# Autodesk Inventor assembly: Pneumatic piston
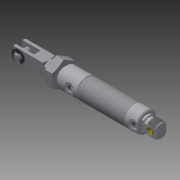
[picture p0: Inventor's stored thumbnail of the model, 180x180]
Saved by Autodesk Inventor 2015 (Build 190159000, 159)
## iProperties
Category: PARTsolutions
Company: BIMBA
Created: 2015-01-25
Part Number: Pneumatic piston
Catalog Web Link: www.cadenas.de
Description: Original Line Standard Air Cylinders-
Vendor: BIMBA
Document SubType Name: Assembly
Designer: chapale16
Manufacturer: BIMBA
PSOL_IDENT_0: {$CADENAS_DATA\23d-libs\bimba\bimba\bimba_imperial\bimba_full_line\original_line_cylinders\standard_
PSOL_IDENT_1: air_cylinders\standard_air_cylinder_asmtab.prj},327 {VTYP=3D},{STYP=ASSTAB},{NB=020.5-DXP(F,D-850)},
PSOL_IDENT_2: {LINA=020.5-DXP},{NN=Original Line Standard Air Cylinders},{DATE=08.09.2014 04:47:41},{GEOMDATE=08.0
PSOL_IDENT_3: 9.2014 04:47:39},{VERSION=},{LINEID=40},{LINESUBID=-1},{WBVAR=STROKE,ACTING,MNT,DER,NR,BM,CO,OO,VO,M
PSOL_IDENT_4: ,EE,EEL,K,Q,Y,G,T,B,H,SER,SR,NT,W,HL,STPT1,STPT2,STPT3,STPT4,MB,PB,PRC,TB,MN}  {NB=020.5-DXP(F,D-850
PSOL_IDENT_5: )},{LINA=020.5-DXP},{KT=DUMMY},{PN=020.5-DXP},{PNC=020.5-DXP(F,D-850)},{PNA=(D-850)},{DASH=-},{BORE1=
PSOL_IDENT_6: 0.56250000},{BORE=9/16\" (02)},{BOREPN=02},{STROKE=0.500},{STROKEALG=[0.011:50/0.001]},{STROKE1=0.50
PSOL_IDENT_7: 0},{ACTING=D},{ACTINGALG= '' , 'Single Acting (SA)' , 'R' , 'Reverse Single Acting (SA)' , 'D' , 'Do
PSOL_IDENT_8: uble Acting (SA)' },{ACTINGPN=D},{MNT=XP},{MNTALG= '' , 'Front Nose Mounting (SA)' , 'XP' , 'Double
PSOL_IDENT_9: End or Rear Pivot Mounting (SA)' , 'X' , 'Double End Mounting (SA)' },{TYPE=},{MNTPN=XP},{DER=},{DER
PSOL_IDENT_10: ALG= '' , 'N/A' },{NR=},{NRALG= '' , 'N/A' },{NRPN=},{BM=},{BMALG= '' , 'N/A' },{BMPN=},{CO=},{COALG=
PSOL_IDENT_11: '' , 'N/A' },{OO=},{OOALG= '', 'N/A' },{OOPN=},{VO=Z},{VOALG= 'Z' , 'N/A' },{VOPN=},{OOVOPN=},{M=},
PSOL_IDENT_12: {MALG= '', 'Without Magnet', 'M', 'With Magnet' },{EE=},{EEL=0.000},{EEMAX=49.5000},{EEALG= '', 'Wit
PSOL_IDENT_13: hout Extra Extension', 'EE', 'With Extra Extension' },{EELALG=0},{EEPN=},{EEPN1=0.000},{K=},{KALG= ''
PSOL_IDENT_14: , 'Standard' , 'K' , 'Ports Rotated 90deg K' },{KPN=},{Q=},{QALG= '' , 'N/A' },{QPN=},{Y=},{YALG= ''
PSOL_IDENT_15: , 'With Pivot Bushing' },{YPN=},{YCON=Y},{F=},{FALG= '', 'Non-Coated (Standard)', 'F', 'Molycoated'
PSOL_IDENT_16: },{FPN=},{G=},{GPN=},{GPN99=},{T=},{TALG= '' , 'Standard -20° to 200°F (-29° to 95°C)' , 'N' , 'Low
PSOL_IDENT_17: Temperature' , 'V' , 'High Temperature' },{NPN=},{VPN=},{B=},{BALG= '', 'W/out Bumpers' , 'B' , 'W/
PSOL_IDENT_18: Bumpers' },{BPN=},{H=},{HALG= '', 'N/A' },{HPN=},{SER=},{SERALG= '' , 'Without Spring Extend/Return'
PSOL_IDENT_19: , 'JS' , 'With Spring Return' , 'JR' , 'With Spring Extend' },{SR=},{SRALG= '' , 'Standard Stainles
PSOL_IDENT_20: s Steel' },{SRPN=},{SRCON=0},{NT=},{NTPN=},{W=},{WALG= '' , 'Without Wiper' , 'W' , 'With Wiper' },{
PSOL_IDENT_21: WPN=},{E=},{EALG= '' , 'Standard Seals/Lube' , 'E' , 'Non-Lube Seals/Lube' },{EPN=},{HL=},{HLALG= ''
PSOL_IDENT_22: , 'Without Low Pressure Hydraulic' , 'HL' , 'With Low Pressure Hydraulic' },{ST=},{STALG= '' , 'N/A'
PSOL_IDENT_23: },{STPT1=},{STPT1ALG= '' , 'N/A' },{STPT2=},{STPT2ALG= '' , 'N/A' },{STPT3=},{STPT3ALG= '' , 'N/A'
PSOL_IDENT_24: },{STPT4=},{STPT4ALG= '' , 'N/A' },{STPN=},{MB=},{MBALG= '' , 'Without Mounting Bracket' , 'F,D-770'
PSOL_IDENT_25: , 'D-770 (front)'  , 'R,D-770' , 'D-770 (rear)' , '2x,D-770' , 'D-770 (front & rear)'},{MBPN=},{MBP
PSOL_IDENT_26: NALL=D-770},{MBPNALLREAR=D-770},{PB=},{PBALG= '' , 'Without Pivot Bracket' , 'D-12321-A' , 'D-12321-
PSOL_IDENT_27: A' },{PBPN=},{PBPNALL=D-12321-A},{PRC=F,D-850},{PRCALG= '' , 'W/out Pivot Rod Clevis' , 'F,D-850' , '
PSOL_IDENT_28: D-850 (front)' },{PRCPN=(F,D-850)},{PRCPNALL=D-850},{TB=},{TBALG= '' , 'N/A' },{TBPN=},{TBPNALL=},{M
PSOL_IDENT_29: N=},{MNALG= '' , 'N/A' },{MNPN=},{MNCONF=},{MNCONR=},{TLEN=1.3870},{FRAC=2.5600},{RGCON=},{RGDACCON=
PSOL_IDENT_30: R},{RHCON=P},{RHCON1=P},{RHCONON=1},{RHACCON=R},{FNUTCON=1},{RNUTCON=1},{FNUTPN=D-154},{RNUTPN=D-154
PSOL_IDENT_31: },{FNUTTRANS=0.0000},{RNUTTRANS=0.0000},{VHOLECON=0},{A1=1.1560},{A1N=1.0310},{A1P=1.1560},{A1B=0.00
PSOL_IDENT_32: 00},{A4=0.1570},{A4N=0.5310},{A4P=0.1570},{A5=0.0250},{A1H=0.969},{A1NH=0.5000},{A1PH=0.9690},{A1BH=
PSOL_IDENT_33: 0.0000},{A1SH=0.0000},{A2H=0.1570},{A2NH=0.1570},{LENGTH=2.5600},{LENGTH1=2.5600},{LENGTH2=2.6100},{
PSOL_IDENT_34: MUL=0.5000},{MUL11=0.5000},{MUL22=1.315},{MUL33=0.8150},{MUL2=0.5000},{MUL211=0.5000},{MUL222=2.6300
PSOL_IDENT_35: },{MUL233=1.6300},{SSS=0.5000},{RGLEN=1.0240},{RHLEN=0.6490},{SSS1=1.0000},{A13=0.7810},{DIF=0.0000}
PSOL_IDENT_36: ,{G5=0.0000},{ON=0},{SSADD=0.0000},{BADD=0.0000},{MADD=0.0000},{NVADD=0.0000},{TRACKL=1.0870},{TRACK
PSOL_IDENT_37: CON=D-74168},{TRIMCON=0},{TRIMCON1=0},{PINCON=},{FSPACE=0.4863},{SPACE=0.0362},{TEXT=0.0633},{S1=0.0
PSOL_IDENT_38: 000},{D1=0.0000},{D1N=0.6150},{D1B=0.6150},{D1P=0.0000},{FA=0.690},{RA=0.6900},{PPATH=standard_air_c
PSOL_IDENT_39: ylinder_asmtpl.prj},{MATALGHTML=<b>Standard Original Line:</b><dl><dt>Rod:</dt><dd>- Stainless Steel
PSOL_IDENT_40: </dd><dd>&nbsp;&nbsp;(5/16 9/16 Bores)</dd><dd>- High Strength Carbon Steel</dd><dd>&nbsp;&nbsp;(3/4
PSOL_IDENT_41: 3 Bore)</dd><dd>- Stainless Steel</dd><dd>&nbsp;&nbsp;(X style DXP/DX/DXDE)</dd><dt>Bearings:</dt><
PSOL_IDENT_42: dd>- Sintered Bronze</dd><dt>Body:</dt><dd>- 304 Stainless Steel</dd><dt>End Caps:</dt><dd>- Aluminu
PSOL_IDENT_43: m</dd><dt>Seals:</dt><dd>- Buna N</dd></dl>},{ASSCFGPRA=02DXP},{MBPNA=},{MNPNA=},{PRCPNA=(D-850)},{A
PSOL_IDENT_44: SSOPTACC=STPT4},{A=3.06},{HADD=0.0000},{WFL=0},{QADD=0.000},{QADD1=0.030},{TEST=0.0000},{MNTB=},{STD
PSOL_IDENT_45: NUTF=1},{STDNUTR=1}
NN: Original Line Standard Air Cylinders
NT: Standard Male Thread
NB: 020.5-DXP(F,D-850)
NBSYN: $PNC.
LINA: 020.5-DXP
PN: 020.5-DXP
PNA: (D-850)
BORE: 9/16" [02]
STROKE: 0.500
ACTING: Double [D]
MNT: Universal Double End or Rear Pivot [XP]
DER: N/A
NR: N/A
BM: N/A
CO: N/A
OO: N/A
VO: N/A
M: Without Magnet Piston
EE: Standard Rod Extension
EEL: 0.000
K: Standard
Q: N/A
Y: Pivot Bushing [Y]
G: Standard Grease Lube
T: Standard -20° to 200°F (-29° to 95°C)
B: Without Bumpers
H: N/A
SER: Without Failsafe Spring Extend/Return
SR: Standard Stainless Steel
W: Without Wiper
HL: Standard 250 PSI Air
STPT1: N/A
STPT2: N/A
STPT3: N/A
STPT4: N/A
MB: Without Mounting Bracket
PB: Without Pivot Bracket
PRC: D-850 (front)
TB: N/A
MN: N/A
A: 3.06
SUPPLIER: BIMBA
ARTICLENO: 020.5-DXP(F,D-850)
BOMINFO: 020.5-DXP
CREATOR: CADENAS GmbH
Title: 020.5-DXP
Author: Cadenas PARTsolutions
## Documents named in this file (13)
- \\lhssvr02\Homedirs\Robotics Club\CAD Model 2015\Elevator parts\Pneumatic piston.iam
- C:\Users\chapale16\Documents\020_5-DXP(F,D-850)0000_0_dummy.ipt
- C:\Users\chapale16\Documents\02R000-0_rod_guide.ipt
- C:\Users\chapale16\Documents\02R-1_3870.ipt
- C:\Users\chapale16\Documents\02P0Y000_rear_head.ipt
- C:\Users\chapale16\Documents\D-154.ipt
- C:\Users\chapale16\Documents\D-8597.ipt
- C:\Users\chapale16\Documents\020_5-DXP0_rod.ipt
- C:\Users\chapale16\Documents\D-850-dummy.ipt
- C:\Users\chapale16\Documents\D-14043.ipt
- C:\Users\chapale16\Documents\D-12304.ipt
- C:\Users\chapale16\Documents\D-5406.ipt
- C:\Users\chapale16\Documents\D-5288.ipt
## Components (13 placed, 12 different names)
1. 020_5-DXP(F,D-850)0000_0_dummy:1 — dummy_XY@1 <-> rod_guide_XY@2, dummy_Z@1 <-> rod_guide_Z@2, dummy_YZ@1 <-> rod_guide_YZ@2
2. 02R000-0_rod_guide:1 — dummy_XY@1 <-> rod_guide_XY@2, dummy_Z@1 <-> rod_guide_Z@2, dummy_YZ@1 <-> rod_guide_YZ@2, to_tube_XY@2 <-> tube_front_XY@3, to_tube_Z@2 <-> tube_front_Z@3, to_tube_YZ@2 <-> tube_front_YZ@3, to_nut_XY@2 <-> NUT_XY@7, to_nut_Z@2 <-> NUT_Z@7, to_nut_YZ@2 <-> NUT_YZ@7, to_rod_XY@2 <-> rod_cp_XY@8, to_rod_Z@2 <-> rod_cp_Z@8
3. 02R-1_3870:1 — to_tube_XY@2 <-> tube_front_XY@3, to_tube_Z@2 <-> tube_front_Z@3, to_tube_YZ@2 <-> tube_front_YZ@3, tube_rear_XY@3 <-> to_tube_XY@4, tube_rear_Z@3 <-> to_tube_Z@4, tube_rear_YZ@3 <-> to_tube_YZ@4
4. 02P0Y000_rear_head:1 — tube_rear_XY@3 <-> to_tube_XY@4, tube_rear_Z@3 <-> to_tube_Z@4, tube_rear_YZ@3 <-> to_tube_YZ@4, to_pin_XY@4 <-> bushing_XY@6, to_pin_Z@4 <-> bushing_Z@6, to_pin_YZ@4 <-> bushing_YZ@6
5. D-8597:1 — to_pin_XY@4 <-> bushing_XY@6, to_pin_Z@4 <-> bushing_Z@6, to_pin_YZ@4 <-> bushing_YZ@6
6. D-154:2 — to_nut_XY@2 <-> NUT_XY@7, to_nut_Z@2 <-> NUT_Z@7, to_nut_YZ@2 <-> NUT_YZ@7
7. 020_5-DXP0_rod:1 — to_rod_XY@2 <-> rod_cp_XY@8, to_rod_Z@2 <-> rod_cp_Z@8, to_rod_clevis_XY@8 <-> to_cyl_XY@9, to_rod_clevis_Z@8 <-> to_cyl_Z@9, to_rod_clevis_YZ@8 <-> to_cyl_YZ@9
8. D-850-dummy:1 — to_rod_clevis_XY@8 <-> to_cyl_XY@9, to_rod_clevis_Z@8 <-> to_cyl_Z@9, to_rod_clevis_YZ@8 <-> to_cyl_YZ@9, dummy_XY@9 <-> dummy_XY@10, dummy_Z@9 <-> dummy_Z@10, dummy_YZ@9 <-> dummy_YZ@10
9. D-14043:1 — dummy_XY@9 <-> dummy_XY@10, dummy_Z@9 <-> dummy_Z@10, dummy_YZ@9 <-> dummy_YZ@10, rod_clevis_body_XY@10 <-> pin_XY@11, rod_clevis_body_Z@10 <-> pin_Z@11, piston_rod_clevis_XY@10 <-> NUT_XY@14, piston_rod_clevis_Z@10 <-> NUT_Z@14
10. D-12304:1 — rod_clevis_body_XY@10 <-> pin_XY@11, rod_clevis_body_Z@10 <-> pin_Z@11, rr1_XY@11 <-> RR_XY@12, rr1_Z@11 <-> RR_Z@12, rr2_XY@11 <-> RR_XY@13, rr2_Z@11 <-> RR_Z@13
11. D-5406:1 — rr1_XY@11 <-> RR_XY@12, rr1_Z@11 <-> RR_Z@12
12. D-5406:2 — rr2_XY@11 <-> RR_XY@13, rr2_Z@11 <-> RR_Z@13
13. D-5288:1 — piston_rod_clevis_XY@10 <-> NUT_XY@14, piston_rod_clevis_Z@10 <-> NUT_Z@14
## Relationships (31: Mate 18, Angle 7, Flush 6)
- dummy_XY@1 <-> rod_guide_XY@2 [Flush]: 020_5-DXP(F,D-850)0000_0_dummy:1 ↔ 02R000-0_rod_guide:1
- dummy_Z@1 <-> rod_guide_Z@2 [Mate]: 020_5-DXP(F,D-850)0000_0_dummy:1 ↔ 02R000-0_rod_guide:1
- dummy_YZ@1 <-> rod_guide_YZ@2 [Angle] (0 deg): 020_5-DXP(F,D-850)0000_0_dummy:1 ↔ 02R000-0_rod_guide:1
- to_tube_XY@2 <-> tube_front_XY@3 [Flush]: 02R000-0_rod_guide:1 ↔ 02R-1_3870:1
- to_tube_Z@2 <-> tube_front_Z@3 [Mate]: 02R000-0_rod_guide:1 ↔ 02R-1_3870:1
- to_tube_YZ@2 <-> tube_front_YZ@3 [Angle] (0 deg): 02R000-0_rod_guide:1 ↔ 02R-1_3870:1
- tube_rear_XY@3 <-> to_tube_XY@4 [Flush]: 02R-1_3870:1 ↔ 02P0Y000_rear_head:1
- tube_rear_Z@3 <-> to_tube_Z@4 [Mate]: 02R-1_3870:1 ↔ 02P0Y000_rear_head:1
- tube_rear_YZ@3 <-> to_tube_YZ@4 [Angle] (0 deg): 02R-1_3870:1 ↔ 02P0Y000_rear_head:1
- to_pin_XY@4 <-> bushing_XY@6 [Mate]: 02P0Y000_rear_head:1 ↔ D-8597:1
- to_pin_Z@4 <-> bushing_Z@6 [Mate]: 02P0Y000_rear_head:1 ↔ D-8597:1
- to_pin_YZ@4 <-> bushing_YZ@6 [Angle] (0 deg): 02P0Y000_rear_head:1 ↔ D-8597:1
- to_nut_XY@2 <-> NUT_XY@7 [Flush]: 02R000-0_rod_guide:1 ↔ D-154:2
- to_nut_Z@2 <-> NUT_Z@7 [Mate]: 02R000-0_rod_guide:1 ↔ D-154:2
- to_nut_YZ@2 <-> NUT_YZ@7 [Angle] (0 deg): 02R000-0_rod_guide:1 ↔ D-154:2
- to_rod_XY@2 <-> rod_cp_XY@8 [Flush]: 02R000-0_rod_guide:1 ↔ 020_5-DXP0_rod:1
- to_rod_Z@2 <-> rod_cp_Z@8 [Mate]: 02R000-0_rod_guide:1 ↔ 020_5-DXP0_rod:1
- to_rod_clevis_XY@8 <-> to_cyl_XY@9 [Flush]: 020_5-DXP0_rod:1 ↔ D-850-dummy:1
- to_rod_clevis_Z@8 <-> to_cyl_Z@9 [Mate]: 020_5-DXP0_rod:1 ↔ D-850-dummy:1
- to_rod_clevis_YZ@8 <-> to_cyl_YZ@9 [Angle] (0 deg): 020_5-DXP0_rod:1 ↔ D-850-dummy:1
- dummy_XY@9 <-> dummy_XY@10 [Mate]: D-850-dummy:1 ↔ D-14043:1
- dummy_Z@9 <-> dummy_Z@10 [Mate]: D-850-dummy:1 ↔ D-14043:1
- dummy_YZ@9 <-> dummy_YZ@10 [Angle] (0 deg): D-850-dummy:1 ↔ D-14043:1
- rod_clevis_body_XY@10 <-> pin_XY@11 [Mate]: D-14043:1 ↔ D-12304:1
- rod_clevis_body_Z@10 <-> pin_Z@11 [Mate]: D-14043:1 ↔ D-12304:1
- rr1_XY@11 <-> RR_XY@12 [Mate]: D-12304:1 ↔ D-5406:1
- rr1_Z@11 <-> RR_Z@12 [Mate]: D-12304:1 ↔ D-5406:1
- rr2_XY@11 <-> RR_XY@13 [Mate]: D-12304:1 ↔ D-5406:2
- rr2_Z@11 <-> RR_Z@13 [Mate]: D-12304:1 ↔ D-5406:2
- piston_rod_clevis_XY@10 <-> NUT_XY@14 [Mate]: D-14043:1 ↔ D-5288:1
- piston_rod_clevis_Z@10 <-> NUT_Z@14 [Mate]: D-14043:1 ↔ D-5288:1
